# Autodesk Inventor assembly: Assembly1
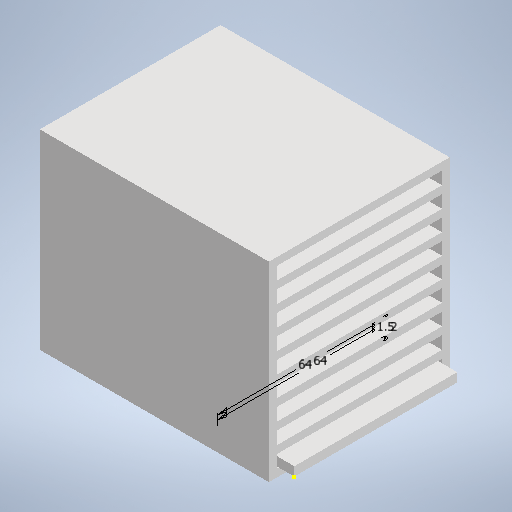
[picture p0: Inventor's stored thumbnail of the model, 512x512]
Saved by Autodesk Inventor 2025.1 (Build 291241020, 241B)
## iProperties
Created: 2024-11-21
Part Number: Assembly1
Document SubType Name: Assembly
Designer: User
Author: User
## Documents named in this file (3)
- C:\Users\User\Documents\Inventor\CardMaster\Assembly1.iam
- C:\Users\User\Documents\Inventor\CardMaster\stack.ipt
- C:\Users\User\Documents\Inventor\CardMaster\shooter.ipt
## Components (2 placed, 2 different names)
1. stack:1 — Mate:1
2. shooter:1 — Mate:1
## Relationships (1: Mate 1)
- Mate:1: stack:1 ↔ shooter:1
